# Autodesk Inventor assembly: TeaTime
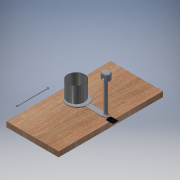
[picture p0: Inventor's stored thumbnail of the model, 180x180]
Saved by Autodesk Inventor 2019 (Build 230136000, 136)
## iProperties
Created: 2020-10-30
Part Number: TeaTime
Document SubType Name: Assembly
Designer: Mike
Author: Mike
## Documents named in this file (7)
- G:\My Drive\Projects\TeaTime\TeaTime.iam
- G:\My Drive\Projects\TeaTime\Mug.ipt
- G:\My Drive\Projects\TeaTime\Table.ipt
- G:\My Drive\Projects\PiCanon\Downloads\raspberry-pi-27.snapshot.7\WEMOS-D1-mini_stl.ipt
- G:\My Drive\Projects\TeaTime\base2.ipt
- G:\My Drive\Projects\TeaTime\fishing_rod.ipt
- G:\My Drive\Projects\TeaTime\top.ipt
## Components (6 placed, 6 different names)
1. Mug:1 — Mate:3
2. Table:1 — Mate:1, Mate:2, Flush:1, Mate:3, Mate:4
3. WEMOS-D1-mini_stl:1
4. base2:1 — Mate:4, Mate:5
5. fishing_rod:1
6. top:1 — Mate:5
## Relationships (6: Mate 5, Flush 1)
- Mate:1: Table:1
- Mate:2: Table:1
- Flush:1: Table:1
- Mate:3: Mug:1 ↔ Table:1
- Mate:4: Table:1 ↔ base2:1
- Mate:5: base2:1 ↔ top:1
